# Autodesk Inventor assembly: Walker Assembly
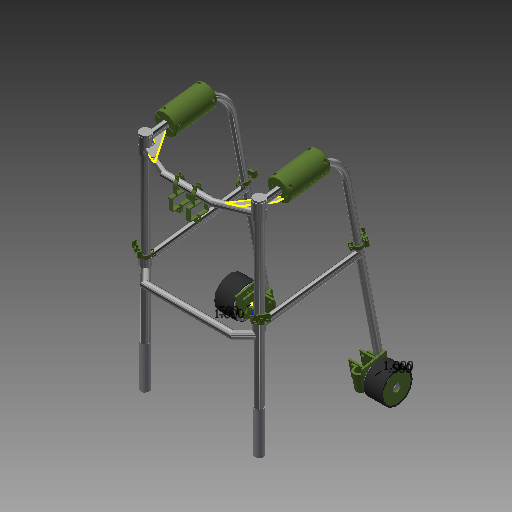
[picture p0: Inventor's stored thumbnail of the model, 512x512]
Saved by Autodesk Inventor 2018 (Build 220112000, 112)
## iProperties
Created: 2018-01-14
Part Number: Walker Assembly
Document SubType Name: Assembly
Designer: prakh
Author: prakh
## Documents named in this file (11)
- D:\GIT\ModernMobility\CADS\Original Walker\Walker Assembly.iam
- D:\GIT\ModernMobility\CADS\Original Walker\front bar.ipt
- D:\GIT\ModernMobility\CADS\Original Walker\Side Rail.ipt
- D:\GIT\ModernMobility\CADS\Original Walker\skid.ipt
- D:\GIT\ModernMobility\CADS\Original Walker\gusset.ipt
- D:\GIT\ModernMobility\CADS\Clutch Wheel compact\Wheel Assembly Left.iam
- D:\GIT\ModernMobility\CADS\Clutch Wheel compact\Wheel Assembly Right.iam
- D:\GIT\ModernMobility\CADS\Sensor Mounts\kinect mount.ipt
- D:\GIT\ModernMobility\CADS\Sensor Mounts\Ultrasonic Mount 1in.ipt
- D:\GIT\ModernMobility\CADS\Sensor Mounts\Ultrasonic Mount 1.14in.ipt
- D:\GIT\ModernMobility\CADS\Handle CADs\Handle Assembly.iam
## Components (17 placed, 10 different names)
1. front bar:1 — Mate:1, Mate:2, Mate:3, Mate:4, Mate:5, Mate:6, Mate:8, Tangent:3, Tangent:5, Mate:9, Tangent:8, Tangent:10, Mate:12, Mate:13, Mate:16, Mate:17
2. Side Rail:1 — Mate:1, Mate:3, Tangent:4, Mate:11, Tangent:11, Tangent:15, Mate:14, Mate:18, Mate:21
3. Side Rail:2 — Mate:2, Mate:4, Tangent:9, Mate:10, Tangent:12, Mate:15, Mate:19, Mate:20
4. skid:1 — Mate:5, Tangent:13
5. skid:2 — Mate:6, Tangent:14
6. gusset:2 — Mate:8, Tangent:3, Tangent:4, Tangent:5
7. gusset:3 — Mate:9, Tangent:8, Tangent:9, Tangent:10
8. Wheel Assembly Left:1 [sub-assembly] — Mate:10, Tangent:12, Tangent:13
9. Wheel Assembly Right:1 [sub-assembly] — Mate:11, Tangent:11, Tangent:14, Tangent:15
10. kinect mount:1 — Mate:12, Flush:1
11. kinect mount:2 — Mate:13, Flush:1
12. Ultrasonic Mount 1in:1 — Mate:14
13. Ultrasonic Mount 1in:2 — Mate:15
14. Ultrasonic Mount 1.14in:1 — Mate:16, Mate:18
15. Ultrasonic Mount 1.14in:2 — Mate:17, Mate:19
16. Handle Assembly:1 [sub-assembly] — Mate:21
17. Handle Assembly:2 [sub-assembly] — Mate:20
## Relationships (32: Mate 20, Tangent 11, Flush 1)
- Mate:1: front bar:1 ↔ Side Rail:1
- Mate:2: front bar:1 ↔ Side Rail:2
- Mate:3: front bar:1 ↔ Side Rail:1
- Mate:4: front bar:1 ↔ Side Rail:2
- Mate:5: front bar:1 ↔ skid:1
- Mate:6: front bar:1 ↔ skid:2
- Mate:8: front bar:1 ↔ gusset:2
- Tangent:3: front bar:1 ↔ gusset:2
- Tangent:4: Side Rail:1 ↔ gusset:2
- Tangent:5 (2.7559 mm): front bar:1 ↔ gusset:2
- Mate:9: front bar:1 ↔ gusset:3
- Tangent:8 (2.7559 mm): front bar:1 ↔ gusset:3
- Tangent:9: Side Rail:2 ↔ gusset:3
- Tangent:10: front bar:1 ↔ gusset:3
- Mate:10: Side Rail:2 ↔ Wheel Assembly Left:1
- Mate:11: Side Rail:1 ↔ Wheel Assembly Right:1
- Tangent:11: Side Rail:1 ↔ Wheel Assembly Right:1
- Tangent:12: Side Rail:2 ↔ Wheel Assembly Left:1
- Tangent:13: skid:1 ↔ Wheel Assembly Left:1
- Tangent:14: skid:2 ↔ Wheel Assembly Right:1
- Tangent:15: Side Rail:1 ↔ Wheel Assembly Right:1
- Mate:12: front bar:1 ↔ kinect mount:1
- Mate:13: front bar:1 ↔ kinect mount:2
- Flush:1: kinect mount:1 ↔ kinect mount:2
- Mate:14: Side Rail:1 ↔ Ultrasonic Mount 1in:1
- Mate:15: Side Rail:2 ↔ Ultrasonic Mount 1in:2
- Mate:16: front bar:1 ↔ Ultrasonic Mount 1.14in:1
- Mate:17: front bar:1 ↔ Ultrasonic Mount 1.14in:2
- Mate:18: Side Rail:1 ↔ Ultrasonic Mount 1.14in:1
- Mate:19: Side Rail:2 ↔ Ultrasonic Mount 1.14in:2
- Mate:20: Side Rail:2 ↔ Handle Assembly:2
- Mate:21: Side Rail:1 ↔ Handle Assembly:1
